# Autodesk Inventor assembly: cameraholder
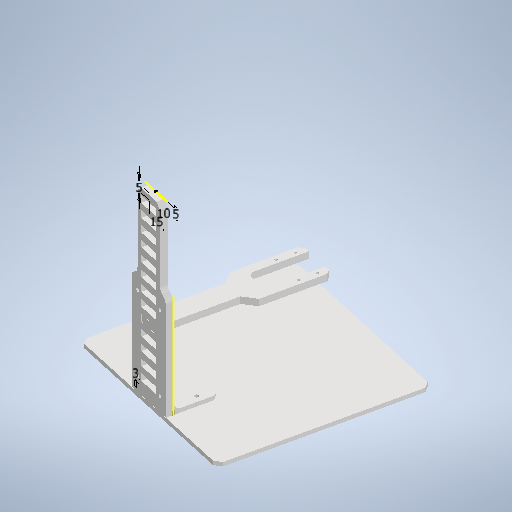
[picture p0: Inventor's stored thumbnail of the model, 512x512]
Saved by Autodesk Inventor 2027 (Build 310192060, 192F)
## iProperties
Created: 2026-05-28
Part Number: cameraholder
Document SubType Name: Assembly
Designer: savas
Author: savas
## Documents named in this file (4)
- C:\Users\savas\Desktop\SWE599\cameraholder.iam
- C:\Users\savas\Desktop\SWE599\ladder.ipt
- C:\Users\savas\Desktop\SWE599\table.ipt
- C:\Users\savas\Desktop\SWE599\camera_holder.ipt
## Components (3 placed, 3 different names)
1. ladder:1 — Mate:2, Mate:3, Mate:4, Flush:1, Mate:5, Mate:6
2. table:1 — Mate:1, Mate:2, Mate:3, Mate:4
3. camera_holder:1 — Flush:1, Mate:5, Mate:6
## Relationships (7: Mate 6, Flush 1)
- Mate:1: table:1
- Mate:2: ladder:1 ↔ table:1
- Mate:3: ladder:1 ↔ table:1
- Mate:4: ladder:1 ↔ table:1
- Flush:1: ladder:1 ↔ camera_holder:1
- Mate:5: ladder:1 ↔ camera_holder:1
- Mate:6: ladder:1 ↔ camera_holder:1
